# Autodesk Inventor assembly: Assembly tandwiel
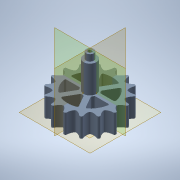
[picture p0: Inventor's stored thumbnail of the model, 180x180]
Saved by Autodesk Inventor 2021 (Build 250183000, 183)
## iProperties
Manager: PJ / DCS
Company: Emmaüs Bovenbouw Aalter
Created: 2021-01-10
Part Number: Assembly tandwiel
Catalog Web Link: http://emmausbovenbouw.op-weg.be/
Vendor: Emmaüs Bovenbouw Aalter
Document SubType Name: Assembly
Designer: Antho
Engineer: Declercq St.
Authority: Declercq St.
Title: Algemene Projecttitel
Author: Antho
## Documents named in this file (3)
- D:\Inventor\GIP 6EM\Assembly\Assembly tandwiel.iam
- D:\Inventor\GIP 6EM\Wielen\Korte as.ipt
- D:\Inventor\GIP 6EM\Wielen\Wiel poging 3.ipt
## Components (2 placed, 2 different names)
1. Korte as:1 — Mate:1, Mate:2, Mate:3
2. Wiel poging 3:1 — Mate:1, Mate:2, Mate:3
## Relationships (3: Mate 3)
- Mate:1: Korte as:1 ↔ Wiel poging 3:1
- Mate:2: Korte as:1 ↔ Wiel poging 3:1
- Mate:3 (0.1 mm): Korte as:1 ↔ Wiel poging 3:1
